# Autodesk Inventor assembly: ArmAssembly
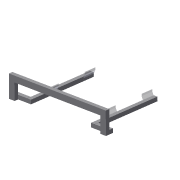
[picture p0: Inventor's stored thumbnail of the model, 180x180]
Saved by Autodesk Inventor 2015 (Build 190159000, 159)
## iProperties
Created: 2015-03-07
Part Number: ArmAssembly
Document SubType Name: Assembly
Designer: Jaden
Author: Jaden
## Documents named in this file (6)
- E:\ReDesign\ArmAssembly.iam
- E:\ReDesign\ArmBar.ipt
- E:\ReDesign\ArmCrossBeam.ipt
- E:\ReDesign\ArmVert.ipt
- E:\ReDesign\armHorzi.ipt
- E:\ReDesign\PChook.ipt
## Components (11 placed, 5 different names)
1. ArmVert:1 — Mate:19, Mate:20, Mate:29, Mate:32
2. ArmVert:2 — Mate:14, Mate:15, Mate:16, Mate:30, Mate:31
3. ArmBar:1 — Mate:17, Mate:18, Mate:23, Flush:1, Mate:24, Flush:2, Flush:3, Mate:25
4. ArmBar:2 — Mate:21, Mate:22, Mate:26, Flush:4, Mate:27, Mate:28, Flush:5, Flush:6
5. armHorzi:1 — Mate:14, Mate:15, Mate:16, Mate:17, Mate:18
6. armHorzi:2 — Mate:19, Mate:20, Mate:21, Mate:22
7. PChook:1 — Mate:26, Flush:4, Mate:27
8. PChook:2 — Mate:28, Flush:5, Flush:6
9. PChook:3 — Mate:24, Flush:2, Flush:3
10. PChook:4 — Mate:23, Flush:1, Mate:25
11. ArmCrossBeam:1 — Mate:29, Mate:30, Mate:31, Mate:32
## Relationships (25: Mate 19, Flush 6)
- Mate:14: ArmVert:2 ↔ armHorzi:1
- Mate:15: ArmVert:2 ↔ armHorzi:1
- Mate:16: ArmVert:2 ↔ armHorzi:1
- Mate:17: ArmBar:1 ↔ armHorzi:1
- Mate:18: ArmBar:1 ↔ armHorzi:1
- Mate:19: ArmVert:1 ↔ armHorzi:2
- Mate:20: ArmVert:1 ↔ armHorzi:2
- Mate:21: ArmBar:2 ↔ armHorzi:2
- Mate:22: ArmBar:2 ↔ armHorzi:2
- Mate:23: ArmBar:1 ↔ PChook:4
- Flush:1 (-6.35 mm): ArmBar:1 ↔ PChook:4
- Mate:24: ArmBar:1 ↔ PChook:3
- Flush:2 (6.35 mm): ArmBar:1 ↔ PChook:3
- Flush:3 (-114.3 mm): ArmBar:1 ↔ PChook:3
- Mate:25: ArmBar:1 ↔ PChook:4
- Mate:26: ArmBar:2 ↔ PChook:1
- Flush:4 (6.35 mm): ArmBar:2 ↔ PChook:1
- Mate:27: ArmBar:2 ↔ PChook:1
- Mate:28: ArmBar:2 ↔ PChook:2
- Flush:5 (114.3 mm): ArmBar:2 ↔ PChook:2
- Flush:6 (6.35 mm): ArmBar:2 ↔ PChook:2
- Mate:29: ArmVert:1 ↔ ArmCrossBeam:1
- Mate:30: ArmVert:2 ↔ ArmCrossBeam:1
- Mate:31: ArmVert:2 ↔ ArmCrossBeam:1
- Mate:32: ArmVert:1 ↔ ArmCrossBeam:1
